# Autodesk Inventor assembly: ASY GBK 3220 central wall shield 5
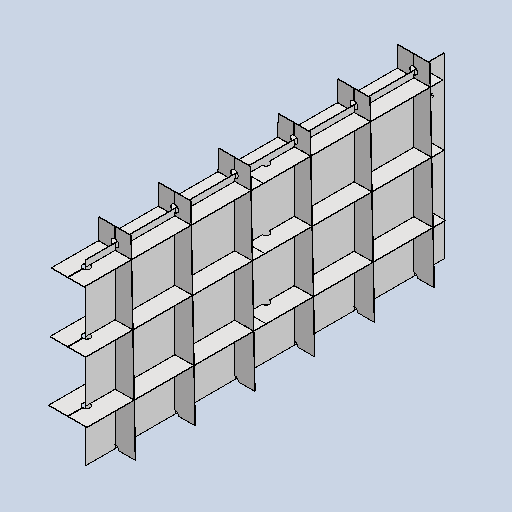
[picture p0: Inventor's stored thumbnail of the model, 512x512]
Saved by Autodesk Inventor 2026.2 (Build 302298010, 298A)
## iProperties
Created: 2026-05-19
Part Number: ASY GBK 3220 central wall shield 5
Document SubType Name: Assembly
Designer: pokla
Mass: 152628 g
Surface Area: 99280.6 cm^2
Volume: 19443.1 cm^3
Density: 7.85 g/cm^3
Author: admin
## Documents named in this file (8)
- C:\Users\admin\Documents\Inventor\GBK-Gubkinskiy\ASY GBK 3220 central wall shield 5.iam
- C:\Users\admin\Documents\Inventor\GBK-Gubkinskiy\GBK 0101 main rib.ipt
- C:\Users\admin\Documents\Inventor\GBK-Gubkinskiy\GBK 3225 shield 5.ipt
- C:\Users\admin\Documents\Inventor\GBK-Gubkinskiy\GBK 3212 central second rib_CPY.ipt
- GBK 3212 central second rib_CPY.ipt
- C:\Users\admin\Documents\Inventor\GBK-Gubkinskiy\GBK 3214 stringer 4.ipt
- C:\Users\admin\Documents\Inventor\GBK-Gubkinskiy\GBK 3215 stringer 5.ipt
- C:\Users\admin\Documents\Inventor\GBK-Gubkinskiy\GBK 3216 stringer 6.ipt
## Components (25 placed, 5 different names)
1. GBK 3214 stringer 4.ipt:1 — Rigid:1, Rigid:10
2. GBK 3215 stringer 5.ipt:1 — Rigid:2, Rigid:11
3. GBK 3216 stringer 6.ipt:1 — Rigid:3, Rigid:12
4. GBK 3214 stringer 4.ipt:2 — Rigid:6, Rigid:7
5. GBK 3215 stringer 5.ipt:2 — Rigid:5, Rigid:8
6. GBK 3216 stringer 6.ipt:2 — Rigid:4, Rigid:9
7. GBK 3225 shield 5.ipt:1 — Flush:6, Mate:7, Mate:8, Mate:6, Flush:8, Flush:7, Mate:5
8. GBK 3214 stringer 4.ipt:3 — Rigid:7
9. GBK 3215 stringer 5.ipt:3 — Rigid:8
10. GBK 3216 stringer 6.ipt:3 — Rigid:9
11. GBK 3214 stringer 4.ipt:4 — Rigid:10
12. GBK 3215 stringer 5.ipt:4 — Rigid:11
13. GBK 3216 stringer 6.ipt:4 — Rigid:12
14. GBK 3212 central second rib_CPY.ipt:1 — Flush:8, Flush:7, Mate:5, Flush:4, Mate:5, Rigid:4, Rigid:5, Rigid:6
15. GBK 3212 central second rib_CPY.ipt:2 — Mate:6, Mate:6, Flush:4, Rigid:3, Rigid:2, Rigid:1
16. GBK 3212 central second rib_CPY.ipt:3
17. GBK 3212 central second rib_CPY.ipt:4
18. GBK 3212 central second rib_CPY.ipt:5
19. GBK 3212 central second rib_CPY.ipt:6
20. GBK 3212 central second rib_CPY.ipt:7
21. GBK 3212 central second rib_CPY.ipt:8
22. GBK 3212 central second rib_CPY.ipt:9
23. GBK 3212 central second rib_CPY.ipt:10
24. GBK 3212 central second rib_CPY.ipt:11
25. GBK 3212 central second rib_CPY.ipt:12
## Component patterns: (6 elements, first: GBK 3212 central second rib_CPY.ipt:1 + GBK 3212 central second rib_CPY.ipt:2)
## Relationships (22: WeldJoint 12, Mate 6, Flush 4)
- Flush:6: GBK 3225 shield 5.ipt:1
- Mate:7: GBK 3225 shield 5.ipt:1
- Mate:8: GBK 3225 shield 5.ipt:1
- Mate:6: GBK 3225 shield 5.ipt:1 ↔ GBK 3212 central second rib_CPY.ipt:2
- Mate:6: GBK 3212 central second rib_CPY.ipt:2
- Flush:8 (250 mm): GBK 3225 shield 5.ipt:1 ↔ GBK 3212 central second rib_CPY.ipt:1
- Flush:7: GBK 3225 shield 5.ipt:1 ↔ GBK 3212 central second rib_CPY.ipt:1
- Mate:5: GBK 3225 shield 5.ipt:1 ↔ GBK 3212 central second rib_CPY.ipt:1
- Flush:4: GBK 3212 central second rib_CPY.ipt:1 ↔ GBK 3212 central second rib_CPY.ipt:2
- Mate:5: GBK 3212 central second rib_CPY.ipt:1
- Rigid:3 [WeldJoint] (4 mm): GBK 3216 stringer 6.ipt:1 ↔ GBK 3212 central second rib_CPY.ipt:2
- Rigid:2 [WeldJoint] (4 mm): GBK 3215 stringer 5.ipt:1 ↔ GBK 3212 central second rib_CPY.ipt:2
- Rigid:1 [WeldJoint] (4 mm): GBK 3214 stringer 4.ipt:1 ↔ GBK 3212 central second rib_CPY.ipt:2
- Rigid:4 [WeldJoint] (4 mm): GBK 3216 stringer 6.ipt:2 ↔ GBK 3212 central second rib_CPY.ipt:1
- Rigid:5 [WeldJoint] (4 mm): GBK 3215 stringer 5.ipt:2 ↔ GBK 3212 central second rib_CPY.ipt:1
- Rigid:6 [WeldJoint] (4 mm): GBK 3214 stringer 4.ipt:2 ↔ GBK 3212 central second rib_CPY.ipt:1
- Rigid:7 [WeldJoint]: GBK 3214 stringer 4.ipt:2 ↔ GBK 3214 stringer 4.ipt:3
- Rigid:8 [WeldJoint]: GBK 3215 stringer 5.ipt:2 ↔ GBK 3215 stringer 5.ipt:3
- Rigid:9 [WeldJoint]: GBK 3216 stringer 6.ipt:2 ↔ GBK 3216 stringer 6.ipt:3
- Rigid:10 [WeldJoint]: GBK 3214 stringer 4.ipt:1 ↔ GBK 3214 stringer 4.ipt:4
- Rigid:11 [WeldJoint]: GBK 3215 stringer 5.ipt:1 ↔ GBK 3215 stringer 5.ipt:4
- Rigid:12 [WeldJoint]: GBK 3216 stringer 6.ipt:1 ↔ GBK 3216 stringer 6.ipt:4
## Named parameters: основание_длина_нижнего = 200 mm, основание_длина_верхнего = 100 mm, стрингер_глубина_1 = 190.70056 mm, стрингер_глубина_2 = 179.35977 mm, стрингер_глубина_3 = 168.01899 mm, стрингер_глубина_4 = 156.6782 mm, стрингер_глубина_5 = 145.33742 mm, стрингер_глубина_6 = 133.99663 mm, стрингер_глубина_7 = 122.65585 mm, стрингер_глубина_8 = 111.31507 mm, Лист_ширина = 1480 mm, ребро_усилителей = 60 mm, паз_под_стрингер_глубина = 70 mm, паз_под_стрингер_толщина = 5 mm, отступ_от_пола_до_первого_стрингера = 410 mm, шаг_стрингеров = 500 mm, радиус_выреза_под_сварку = 30 mm, нахлест_шпангоутов_1_2 = 150 mm, нахлест_шпангоутов_2_3 = 120 mm, Стрингер_длина = 1489.5 mm, Лист_длина = 2980 mm, Шаг_шпангоутов = 496.66667 mm
